# Autodesk Inventor assembly: Assembly1
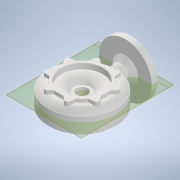
[picture p0: Inventor's stored thumbnail of the model, 180x180]
Saved by Autodesk Inventor 2020 (Build 240168000, 168)
## iProperties
Created: 2020-08-16
Part Number: Assembly1
Document SubType Name: Assembly
Designer: benny
Author: benny
## Documents named in this file (3)
- C:\Users\benny\Desktop\importantmajorprojecthev_june\New folder\Assembly1.iam
- C:\Users\benny\Desktop\importantmajorprojecthev_june\New folder\Part2.ipt
- C:\Users\benny\Desktop\importantmajorprojecthev_june\New folder\suction casting machine.ipt
## Components (2 placed, 2 different names)
1. Part2:1 — Mate:1, Mate:2, Mate:3
2. suction casting machine:1 — Mate:1, Mate:2, Mate:3, Flush:1, Mate:4, Mate:5
## Relationships (6: Mate 5, Flush 1)
- Mate:1: Part2:1 ↔ suction casting machine:1
- Mate:2: Part2:1 ↔ suction casting machine:1
- Mate:3: Part2:1 ↔ suction casting machine:1
- Flush:1: suction casting machine:1
- Mate:4: suction casting machine:1
- Mate:5: suction casting machine:1
